# Autodesk Inventor assembly: Assembly1
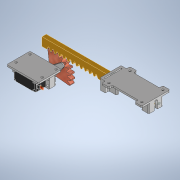
[picture p0: Inventor's stored thumbnail of the model, 180x180]
Saved by Autodesk Inventor 2022 (Build 260153000, 153)
## iProperties
Created: 2022-06-04
Part Number: Assembly1
Document SubType Name: Assembly
Designer: frede
Author: frede
## Documents named in this file (10)
- C:\Users\frede\OneDrive\Desktop\DigCow\Assembly1.iam
- C:\Users\frede\Downloads\Servo Motor MG996R.ipt
- C:\Users\frede\OneDrive\Desktop\DigCow\Rack222.ipt
- C:\Users\frede\OneDrive\Desktop\DigCow\Pinion222.ipt
- C:\Users\frede\OneDrive\Desktop\DigCow\Syringe.ipt
- C:\Users\frede\OneDrive\Desktop\DigCow\RackSlider.ipt
- C:\Users\frede\OneDrive\Documents\Inventor\Content Center Files\R2022\en-US\DIN 912\DIN 912 - M3 x 0.5 x 10 x 8.75.ipt
- C:\Users\frede\OneDrive\Desktop\DigCow\MotorCasingSmall.ipt
- C:\Users\frede\OneDrive\Desktop\DigCow\SyringeCasing.ipt
- C:\Users\frede\OneDrive\Documents\NyArm.ipt
## Components (9 placed, 9 different names)
1. Servo Motor MG996R:1 — Angle:2, Flush:2, Angle:3, Flush:3, Flush:4, Insert:4, Mate:3
2. Rack222:1 — Flush:1, Angle:2, Flush:2, Rotation/Translation:1, Insert:2, Mate:1, Mate:2
3. Pinion222:1 — Flush:1, Rotation/Translation:1, Rotation:1, Mate:3, Insert:5, Angle:4
4. Syringe:1 — Insert:2, Angle:3
5. RackSlider:1 — Mate:1, Mate:2, Flush:3, Flush:5
6. DIN 912 - replaced by DIN EN ISO 4762 M3 x 10:1 — Rotation:1, Insert:5
7. MotorCasingSmall:1 — Flush:4
8. SyringeCasing:1 — Flush:5
9. NyArm:1 — Insert:4, Angle:4
## Relationships (16: Flush 5, Angle 3, Insert 3, Mate 3, RelateRotateTranslate 1, RelateRotation 1)
- Flush:1: Rack222:1 ↔ Pinion222:1
- Angle:2 (0 deg): Servo Motor MG996R:1 ↔ Rack222:1
- Flush:2 (32.6 mm): Servo Motor MG996R:1 ↔ Rack222:1
- Rotation/Translation:1 [RelateRotateTranslate] (183 mm): Rack222:1 ↔ Pinion222:1
- Insert:2 (1.5 mm): Rack222:1 ↔ Syringe:1
- Angle:3 (0 deg): Servo Motor MG996R:1 ↔ Syringe:1
- Mate:1 (0.1 mm): Rack222:1 ↔ RackSlider:1
- Mate:2 (0.5 mm): Rack222:1 ↔ RackSlider:1
- Flush:3 (53 mm): Servo Motor MG996R:1 ↔ RackSlider:1
- Rotation:1 [RelateRotation] (1 ul): Pinion222:1 ↔ DIN 912 - replaced by DIN EN ISO 4762 M3 x 10:1
- Flush:4: Servo Motor MG996R:1 ↔ MotorCasingSmall:1
- Flush:5: RackSlider:1 ↔ SyringeCasing:1
- Insert:4: Servo Motor MG996R:1 ↔ NyArm:1
- Mate:3: Servo Motor MG996R:1 ↔ Pinion222:1
- Insert:5: Pinion222:1 ↔ DIN 912 - replaced by DIN EN ISO 4762 M3 x 10:1
- Angle:4 (180 deg): Pinion222:1 ↔ NyArm:1
